# Autodesk Inventor assembly: TheClaw
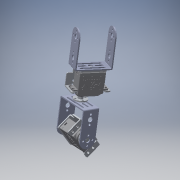
[picture p0: Inventor's stored thumbnail of the model, 180x180]
Saved by Autodesk Inventor 2017 (Build 210142000, 142)
## iProperties
Created: 2017-09-30
Part Number: TheClaw
Document SubType Name: Assembly
Designer: User
Author: User
## Documents named in this file (5)
- C:\Robotics\CAD\2017-18_CAD\TheClaw.iam
- C:\Robotics\CAD\COTSParts\Tetrix\39593_txm-standard-scale pivot armwbearing..ipt
- C:\Robotics\CAD\COTSParts\Tetrix\39020_txm-servo mount horn.ipt
- C:\Robotics\CAD\COTSParts\Vex\REV-41-1097.ipt
- C:\Robotics\CAD\COTSParts\Tetrix\39060_txm-standard servo bracket.ipt
## Components (8 placed, 4 different names)
1. 39593_txm-standard-scale pivot armwbearing.:1 — Mate:16, Mate:17, Mate:18, Mate:25, Mate:26
2. 39020_txm-servo mount horn:1 — Mate:16, Mate:17, Mate:18, Mate:23, Mate:24
3. 39020_txm-servo mount horn:2 — Mate:25, Mate:26, Mate:27, Mate:28
4. REV-41-1097:2 — Mate:19, Mate:20, Mate:21, Mate:22, Mate:23, Mate:24
5. REV-41-1097:3 — Mate:27, Mate:28, Mate:30, Mate:31, Mate:34
6. 39593_txm-standard-scale pivot armwbearing.:2 — Mate:32, Mate:33, Flush:1
7. 39060_txm-standard servo bracket:1 — Mate:19, Mate:20, Mate:21, Mate:22
8. 39060_txm-standard servo bracket:2 — Mate:30, Mate:31, Mate:32, Mate:33, Mate:34, Flush:1
## Relationships (19: Mate 18, Flush 1)
- Mate:16 (3.6322 mm): 39593_txm-standard-scale pivot armwbearing.:1 ↔ 39020_txm-servo mount horn:1
- Mate:17 (3.6322 mm): 39593_txm-standard-scale pivot armwbearing.:1 ↔ 39020_txm-servo mount horn:1
- Mate:18 (3.6322 mm): 39593_txm-standard-scale pivot armwbearing.:1 ↔ 39020_txm-servo mount horn:1
- Mate:19: REV-41-1097:2 ↔ 39060_txm-standard servo bracket:1
- Mate:20: REV-41-1097:2 ↔ 39060_txm-standard servo bracket:1
- Mate:21: REV-41-1097:2 ↔ 39060_txm-standard servo bracket:1
- Mate:22: REV-41-1097:2 ↔ 39060_txm-standard servo bracket:1
- Mate:23: 39020_txm-servo mount horn:1 ↔ REV-41-1097:2
- Mate:24: 39020_txm-servo mount horn:1 ↔ REV-41-1097:2
- Mate:25 (3.6322 mm): 39593_txm-standard-scale pivot armwbearing.:1 ↔ 39020_txm-servo mount horn:2
- Mate:26: 39593_txm-standard-scale pivot armwbearing.:1 ↔ 39020_txm-servo mount horn:2
- Mate:27: 39020_txm-servo mount horn:2 ↔ REV-41-1097:3
- Mate:28: 39020_txm-servo mount horn:2 ↔ REV-41-1097:3
- Mate:30: REV-41-1097:3 ↔ 39060_txm-standard servo bracket:2
- Mate:31: REV-41-1097:3 ↔ 39060_txm-standard servo bracket:2
- Mate:32: 39593_txm-standard-scale pivot armwbearing.:2 ↔ 39060_txm-standard servo bracket:2
- Mate:33: 39593_txm-standard-scale pivot armwbearing.:2 ↔ 39060_txm-standard servo bracket:2
- Mate:34: REV-41-1097:3 ↔ 39060_txm-standard servo bracket:2
- Flush:1 (8.001 mm): 39593_txm-standard-scale pivot armwbearing.:2 ↔ 39060_txm-standard servo bracket:2
